# Autodesk Inventor assembly: drive tensioner
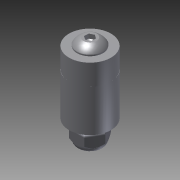
[picture p0: Inventor's stored thumbnail of the model, 180x180]
Saved by Autodesk Inventor 2014 SP1 (Build 180222100, 222)
## iProperties
Created: 2013-10-24
Part Number: drive tensioner
Document SubType Name: Assembly
Designer: RyanHughes
Author: RyanHughes
## Documents named in this file (6)
- C:\Users\Ryan\Desktop\sw\toss up 2ed A bot\drivetrain\drive tensioner.iam
- C:\Users\Ryan\Desktop\sw\lib\Aperture VEX CAD Library\Spacers\SPACER-0500-0500.ipt
- C:\Users\Ryan\Desktop\sw\lib\Aperture VEX CAD Library\Hardware\8-32\8-32 Nylock.ipt
- C:\Users\Ryan\Desktop\sw\lib\Aperture VEX CAD Library\Sprockets\HS Sprockets\High strength Chain Link.ipt
- C:\Users\Ryan\Desktop\sw\lib\Aperture VEX CAD Library\Spacers\SPACER-0500-0250.ipt
- C:\Users\Ryan\Desktop\sw\lib\Aperture VEX CAD Library\Hardware\8-32\8-32_1.000.ipt
## Components (5 placed, 5 different names)
1. SPACER-0500-0500:1 — Mate:1, Mate:2, Tangent:1, Mate:5, Mate:6
2. 8-32_1.000:1 — Mate:7
3. 8-32 Nylock:1 — Mate:6, Mate:7
4. High strength Chain Link:1 — Tangent:1, Mate:5
5. SPACER-0500-0250:1 — Mate:1, Mate:2
## Relationships (8: Mate 7, Tangent 1)
- Mate:1: SPACER-0500-0500:1 ↔ SPACER-0500-0250:1
- Mate:2: SPACER-0500-0500:1 ↔ SPACER-0500-0250:1
- [Mate]: 8-32_1.000:1 ↔ SPACER-0500-0250:1
- [Mate]: SPACER-0500-0500:1 ↔ 8-32_1.000:1
- Tangent:1: SPACER-0500-0500:1 ↔ High strength Chain Link:1
- Mate:5: SPACER-0500-0500:1 ↔ High strength Chain Link:1
- Mate:6 (1.5875 mm): SPACER-0500-0500:1 ↔ 8-32 Nylock:1
- Mate:7: 8-32_1.000:1 ↔ 8-32 Nylock:1
